# Autodesk Inventor assembly: sestava tělo estonsko s plechem
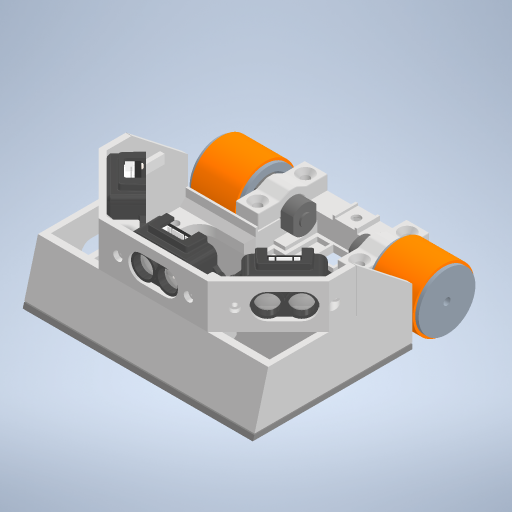
[picture p0: Inventor's stored thumbnail of the model, 512x512]
Saved by Autodesk Inventor 2024 (Build 280153000, 153)
## iProperties
Created: 2023-11-06
Part Number: sestava tělo estonsko s plechem
Document SubType Name: Assembly
Designer: jaryj
Author: jaryj
## Documents named in this file (8)
- C:\Users\Simak\OneDrive\Dokumenty\GitHub\RoboCop\- 3D -\wip\Tělo s plechem\sestava tělo estonsko s plechem.iam
- C:\Users\Simak\OneDrive\Dokumenty\GitHub\RoboCop\- 3D -\wip\Tělo s plechem\Plech.ipt
- C:\Users\Simak\OneDrive\Dokumenty\GitHub\RoboCop\- 3D -\wip\Tělo s plechem\tělo estonsko s plechem.ipt
- C:\Users\Simak\OneDrive\Dokumenty\GitHub\RoboCop\- 3D -\el._parts\GA12-N20_Motor.ipt
- C:\Users\Simak\OneDrive\Dokumenty\GitHub\RoboCop\- 3D -\mech._parts\motor_C_clamp.ipt
- C:\Users\Simak\OneDrive\Dokumenty\GitHub\RoboCop\- 3D -\mech._parts\wheel+silicon.ipt
- C:\Users\Simak\OneDrive\Dokumenty\GitHub\RoboCop\- 3D -\el._parts\sumec\sumec.ipt
- C:\Users\Simak\OneDrive\Dokumenty\GitHub\RoboCop\- 3D -\wip\Sestava TF-Luna a držáku.iam
## Components (10 placed, 7 different names)
1. Plech:1 — Rotační:1, Vložit:1
2. tělo estonsko s plechem:1 — Rotační:1, Vložit:1, Vložit:2, Proti sobě:1, Vložit:3, Proti sobě:2, Proti sobě:5, Proti sobě:6, Vložit:4, Vložit:5, Proti sobě:9, Vložit:6, Vložit:7, Proti sobě:10, Stejný směr:1, Proti sobě:11
3. GA12-N20_Motor:1 — Vložit:2, Proti sobě:1, Proti sobě:3, Proti sobě:8
4. GA12-N20_Motor:2 — Vložit:3, Proti sobě:2, Proti sobě:4, Proti sobě:7
5. motor_C_clamp:1 — Proti sobě:8, Vložit:5
6. wheel+silicon:1 — Proti sobě:4, Proti sobě:5
7. motor_C_clamp:2 — Proti sobě:7, Vložit:4
8. wheel+silicon:2 — Proti sobě:3, Proti sobě:6
9. sumec:1 — Proti sobě:9, Vložit:6, Vložit:7
10. Sestava TF-Luna a držáku:1 [sub-assembly] — Proti sobě:10, Stejný směr:1, Proti sobě:11
## Relationships (20: Mate 11, Insert 7, RevoluteJoint 1, Flush 1)
- Rotační:1 [RevoluteJoint]: Plech:1 ↔ tělo estonsko s plechem:1
- Vložit:1 [Insert]: Plech:1 ↔ tělo estonsko s plechem:1
- Vložit:2 [Insert]: tělo estonsko s plechem:1 ↔ GA12-N20_Motor:1
- Proti sobě:1 [Mate]: tělo estonsko s plechem:1 ↔ GA12-N20_Motor:1
- Vložit:3 [Insert]: tělo estonsko s plechem:1 ↔ GA12-N20_Motor:2
- Proti sobě:2 [Mate]: tělo estonsko s plechem:1 ↔ GA12-N20_Motor:2
- Proti sobě:3 [Mate]: GA12-N20_Motor:1 ↔ wheel+silicon:2
- Proti sobě:4 [Mate]: GA12-N20_Motor:2 ↔ wheel+silicon:1
- Proti sobě:5 [Mate] (0.5 mm): tělo estonsko s plechem:1 ↔ wheel+silicon:1
- Proti sobě:6 [Mate] (0.5 mm): tělo estonsko s plechem:1 ↔ wheel+silicon:2
- Proti sobě:7 [Mate]: GA12-N20_Motor:2 ↔ motor_C_clamp:2
- Vložit:4 [Insert]: tělo estonsko s plechem:1 ↔ motor_C_clamp:2
- Proti sobě:8 [Mate]: GA12-N20_Motor:1 ↔ motor_C_clamp:1
- Vložit:5 [Insert]: tělo estonsko s plechem:1 ↔ motor_C_clamp:1
- Proti sobě:9 [Mate]: tělo estonsko s plechem:1 ↔ sumec:1
- Vložit:6 [Insert]: tělo estonsko s plechem:1 ↔ sumec:1
- Vložit:7 [Insert]: tělo estonsko s plechem:1 ↔ sumec:1
- Proti sobě:10 [Mate]: tělo estonsko s plechem:1 ↔ Sestava TF-Luna a držáku:1
- Stejný směr:1 [Flush]: tělo estonsko s plechem:1 ↔ Sestava TF-Luna a držáku:1
- Proti sobě:11 [Mate] (-11.1058 mm): tělo estonsko s plechem:1 ↔ Sestava TF-Luna a držáku:1
